# Autodesk Inventor assembly: draft1
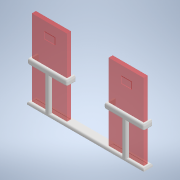
[picture p0: Inventor's stored thumbnail of the model, 180x180]
Saved by Autodesk Inventor 2020 (Build 240168000, 168)
## iProperties
Created: 2020-03-06
Part Number: draft1
Document SubType Name: Assembly
Designer: Sverrir
Author: Sverrir
## Documents named in this file (3)
- C:\Users\Sverrir\Desktop\Skóli\Human-Centered Artificial Intelligence\1. Semester\Computer vision\Project\3D\draft1.iam
- C:\Users\Sverrir\Desktop\Skóli\Human-Centered Artificial Intelligence\1. Semester\Computer vision\Project\3D\Mount&holder.ipt
- C:\Users\Sverrir\Desktop\Skóli\Human-Centered Artificial Intelligence\1. Semester\Computer vision\Project\3D\galaxy s8 dimensions.ipt
## Components (3 placed, 2 different names)
1. Mount&holder:1 — Mate:1, Mate:2, Mate:3, Mate:4, Mate:5, Mate:6
2. galaxy s8 dimensions:1 — Mate:3, Mate:4, Mate:5
3. galaxy s8 dimensions:2 — Mate:1, Mate:2, Mate:6
## Relationships (6: Mate 6)
- Mate:1: Mount&holder:1 ↔ galaxy s8 dimensions:2
- Mate:2: Mount&holder:1 ↔ galaxy s8 dimensions:2
- Mate:3: Mount&holder:1 ↔ galaxy s8 dimensions:1
- Mate:4: Mount&holder:1 ↔ galaxy s8 dimensions:1
- Mate:5: Mount&holder:1 ↔ galaxy s8 dimensions:1
- Mate:6: Mount&holder:1 ↔ galaxy s8 dimensions:2
